# Autodesk Inventor assembly: subassembly_auger_case
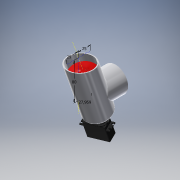
[picture p0: Inventor's stored thumbnail of the model, 180x180]
Saved by Autodesk Inventor 2019 (Build 230136000, 136)
## iProperties
Created: 2019-01-23
Part Number: subassembly_auger_case
Document SubType Name: Assembly
Designer: jmc
Author: jmc
## Documents named in this file (5)
- D:\Inventor\Projects\CatFeeder\version4 (auger)\subassembly_auger_case.iam
- D:\Inventor\Projects\CatFeeder\Auger\auger.ipt
- D:\Inventor\Projects\CatFeeder\Auger\screw.ipt
- D:\Inventor\Projects\3party\Servos\MG995.ipt
- D:\Inventor\Projects\CatFeeder\Auger\servo_adapter.ipt
## Components (4 placed, 4 different names)
1. auger:1 — Rotational:1
2. screw:1 — Rotational:1, Rigid:1
3. MG995:1 — Rigid:2
4. servo_adapter:1 — Rigid:1, Rigid:2
## Relationships (3: WeldJoint 2, RevoluteJoint 1)
- Rotational:1 [RevoluteJoint]: auger:1 ↔ screw:1
- Rigid:1 [WeldJoint]: screw:1 ↔ servo_adapter:1
- Rigid:2 [WeldJoint]: MG995:1 ↔ servo_adapter:1
